# Autodesk Inventor assembly: Coil Designs
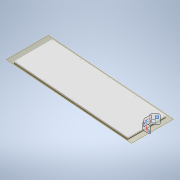
[picture p0: Inventor's stored thumbnail of the model, 180x180]
Saved by Autodesk Inventor 2021 (Build 250183000, 183)
## iProperties
Created: 2022-01-19
Part Number: Coil Designs
Document SubType Name: Assembly
Designer: avan411
Author: avan411
## Documents named in this file (9)
- H:\GitRepos\2021_SRW_RC_CAR\Magnetics\Tested coil designs\DoubleD\CadModels\Coil Designs.iam
- H:\GitRepos\2021_SRW_RC_CAR\Magnetics\Tested coil designs\DoubleD\CadModels\FerriteBar.ipt
- H:\GitRepos\2021_SRW_RC_CAR\Magnetics\Tested coil designs\DoubleD\CadModels\Part2.ipt
- H:\GitRepos\2021_SRW_RC_CAR\Magnetics\Tested coil designs\DoubleD\CadModels\PrimaryCoilFerriteLayer.ipt
- \\unifiles.uoa.auckland.ac.nz\myhome\Documents\btwnFerriteAndCoil.ipt
- \\unifiles.uoa.auckland.ac.nz\myhome\Documents\between aluminium and ferrite.ipt
- H:\GitRepos\2021_SRW_RC_CAR\Magnetics\Tested coil designs\DoubleD\CadModels\PrimaryCoilAluminiumLayer.ipt
- \\unifiles.uoa.auckland.ac.nz\myhome\Documents\aluminium.ipt
- \\unifiles.uoa.auckland.ac.nz\myhome\Documents\base.ipt
## Components (25 placed, 8 different names)
1. PrimaryCoilLayer:1 — Flush:1
2. btwnFerriteAndCoil:1 — Flush:1, Mate:3, Flush:2, Flush:3, Flush:4
3. PrimaryCoifERRITElLayer:2 — Mate:3, Flush:2, Flush:3, Flush:5, Flush:6
4. between aluminium and ferrite:1 — Flush:6, Flush:7, Flush:8, Mate:4, Flush:9, Flush:10
5. PrimaryCoiAluminiumlLayer:3 — Flush:7, Flush:8, Mate:4, Flush:11, Flush:12, Mate:5
6. aluminium:1 — Flush:9, Flush:10
7. base:1 — Flush:11, Flush:12, Mate:5
8. FerriteBar:2 — Mate:1, Mate:2
9. FerriteBar:1 — Mate:1, Mate:2, Flush:4, Flush:5
10. FerriteBar:3
11. FerriteBar:4
12. FerriteBar:5
13. FerriteBar:6
14. FerriteBar:7
15. FerriteBar:8
16. FerriteBar:9
17. FerriteBar:10
18. FerriteBar:11
19. FerriteBar:12
20. FerriteBar:13
21. FerriteBar:14
22. FerriteBar:15
23. FerriteBar:16
24. FerriteBar:17
25. FerriteBar:18
## Component patterns: (9 elements, first: FerriteBar:2 + FerriteBar:1)
## Relationships (17: Flush 12, Mate 5)
- Mate:1: FerriteBar:2 ↔ FerriteBar:1
- Mate:2: FerriteBar:2 ↔ FerriteBar:1
- Flush:1: PrimaryCoilLayer:1 ↔ btwnFerriteAndCoil:1
- Mate:3: btwnFerriteAndCoil:1 ↔ PrimaryCoifERRITElLayer:2
- Flush:2: btwnFerriteAndCoil:1 ↔ PrimaryCoifERRITElLayer:2
- Flush:3: btwnFerriteAndCoil:1 ↔ PrimaryCoifERRITElLayer:2
- Flush:4 (-60 mm): btwnFerriteAndCoil:1 ↔ FerriteBar:1
- Flush:5: PrimaryCoifERRITElLayer:2 ↔ FerriteBar:1
- Flush:6: PrimaryCoifERRITElLayer:2 ↔ between aluminium and ferrite:1
- Flush:7: between aluminium and ferrite:1 ↔ PrimaryCoiAluminiumlLayer:3
- Flush:8: between aluminium and ferrite:1 ↔ PrimaryCoiAluminiumlLayer:3
- Mate:4: between aluminium and ferrite:1 ↔ PrimaryCoiAluminiumlLayer:3
- Flush:9: between aluminium and ferrite:1 ↔ aluminium:1
- Flush:10: between aluminium and ferrite:1 ↔ aluminium:1
- Flush:11: PrimaryCoiAluminiumlLayer:3 ↔ base:1
- Flush:12: PrimaryCoiAluminiumlLayer:3 ↔ base:1
- Mate:5: PrimaryCoiAluminiumlLayer:3 ↔ base:1
